# Autodesk Inventor assembly: Assembly1
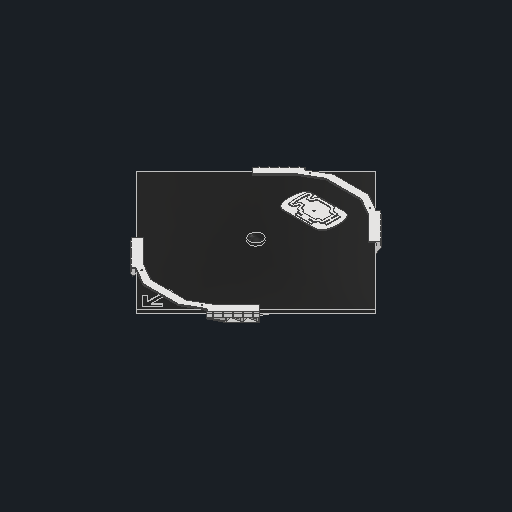
[picture p0: Inventor's stored thumbnail of the model, 512x512]
Saved by Autodesk Inventor 2026 (Build 300175050, 175E)
## iProperties
Created: 2025-05-29
Part Number: Assembly1
Document SubType Name: Assembly
Designer: Natha
Author: Natha
## Documents named in this file (9)
- C:\Users\Natha\Desktop\Grad Cap\cad\Assembly1.iam
- C:\Users\Natha\OneDrive\Documents\Cap.ipt
- C:\Users\Natha\Desktop\Grad Cap\cad\front_lights.ipt
- C:\Users\Natha\Desktop\Grad Cap\cad\electronics.ipt
- C:\Users\Natha\Desktop\Grad Cap\cad\new_electronics_box.ipt
- C:\Users\Natha\Desktop\Grad Cap\cad\battery_box.ipt
- C:\Users\Natha\Desktop\Grad Cap\cad\power_switch.ipt
- C:\Users\Natha\Desktop\Grad Cap\cad\engine _light.ipt
- C:\Users\Natha\Desktop\Grad Cap\cad\new_power_switch.ipt
## Components (8 placed, 8 different names)
1. Cap:1 — Flush:8
2. front_rear_lights:1 — Flush:2, Flush:3
3. electronics rev 1 — Flush:4
4. new_electronics_box:1 — Flush:5
5. battery_box:1 — Flush:6
6. power_switch:1 — Flush:7
7. engine _light:1 — Flush:8
8. new_power_switch:1 — Flush:9
## Relationships (9: Flush 9)
- Flush:1 (5 mm)
- Flush:2: front_rear_lights:1
- Flush:3: front_rear_lights:1
- Flush:4: electronics rev 1
- Flush:5: new_electronics_box:1
- Flush:6: battery_box:1
- Flush:7: power_switch:1
- Flush:8: Cap:1 ↔ engine _light:1
- Flush:9: new_power_switch:1
